# Autodesk Inventor assembly: GenevaDrive
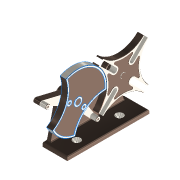
[picture p0: Inventor's stored thumbnail of the model, 180x180]
Saved by Autodesk Inventor 2022.2 (Build 262287010, 287A)
## iProperties
Created: 2022-12-22
Part Number: GenevaDrive
Document SubType Name: Assembly
Designer: User
Author: User
## Documents named in this file (9)
- C:\Users\User\Desktop\InventorTutorial prof Stancesu\Part18 Geneva drive Components\GenevaDrive.iam
- C:\Users\User\Desktop\InventorTutorial prof Stancesu\Part18 Geneva drive Components\Support.ipt
- C:\Users\User\Desktop\InventorTutorial prof Stancesu\Part18 Geneva drive Components\Lever.ipt
- C:\Users\User\Desktop\InventorTutorial prof Stancesu\Part18 Geneva drive Components\Axle Big.ipt
- C:\Users\User\Desktop\InventorTutorial prof Stancesu\Part18 Geneva drive Components\Axle Small.ipt
- C:\Users\User\Desktop\InventorTutorial prof Stancesu\Part18 Geneva drive Components\Disk.ipt
- C:\Users\User\Desktop\InventorTutorial prof Stancesu\Part18 Geneva drive Components\Malta Cross.ipt
- C:\Users\User\Desktop\InventorTutorial prof Stancesu\Part18 Geneva drive Components\Roller.ipt
- C:\Users\User\Desktop\InventorTutorial prof Stancesu\Part18 Geneva drive Components\Pin.ipt
## Components (12 placed, 8 different names)
1. Support:1 — Mate:1, Flush:1, Insert:1, Insert:2, Insert:3, Angle:1
2. Lever:1 — Insert:2, Insert:4, Insert:5, Insert:6, Insert:7, Insert:8, Mate:2, Mate:3, Angle:1
3. Axle Big:1 — Mate:1, Flush:1
4. Axle Big:2 — Insert:1
5. Axle Small:1 — Insert:5
6. Axle Small:2 — Insert:7
7. Disk:1 — Insert:4, Mate:2, Mate:3, Insert:9, Insert:10
8. Malta Cross:1 — Insert:3
9. Roller:1 — Insert:8
10. Roller:2 — Insert:6
11. Pin:1 — Insert:10
12. Pin:2 — Insert:9
## Relationships (15: Insert 10, Mate 3, Flush 1, Angle 1)
- Mate:1: Support:1 ↔ Axle Big:1
- Flush:1: Support:1 ↔ Axle Big:1
- Insert:1: Support:1 ↔ Axle Big:2
- Insert:2: Support:1 ↔ Lever:1
- Insert:3: Support:1 ↔ Malta Cross:1
- Insert:4: Lever:1 ↔ Disk:1
- Insert:5: Lever:1 ↔ Axle Small:1
- Insert:6: Lever:1 ↔ Roller:2
- Insert:7: Lever:1 ↔ Axle Small:2
- Insert:8: Lever:1 ↔ Roller:1
- Mate:2: Lever:1 ↔ Disk:1
- Mate:3: Lever:1 ↔ Disk:1
- Insert:9: Disk:1 ↔ Pin:2
- Insert:10: Disk:1 ↔ Pin:1
- Angle:1 (0 deg): Support:1 ↔ Lever:1
